# Autodesk Inventor assembly: Assembly
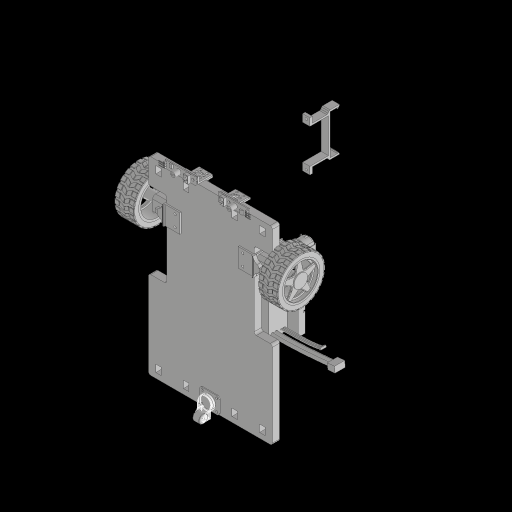
[picture p0: Inventor's stored thumbnail of the model, 512x512]
Saved by Autodesk Inventor 2024.3 (Build 283343010, 343A)
## iProperties
Created: 2025-04-09
Part Number: Assembly
Document SubType Name: Assembly
Designer: Oleg Kelner
Author: Oleg Kelner
## Documents named in this file (14)
- D:\Study\Prototyping\Prototyping-SS25-Team-C4\3DModels\Assembly.iam
- D:\Study\Prototyping\Prototyping-SS25-Team-C4\3DModels\Basic components\chassis.ipt
- D:\Study\Prototyping\Prototyping-SS25-Team-C4\3DModels\Basic components\motor-with-tire.ipt
- D:\Study\Prototyping\Prototyping-SS25-Team-C4\3DModels\Basic components\front-wheel.ipt
- D:\Study\Prototyping\Prototyping-SS25-Team-C4\3DModels\Basic components\motor-with-tire_MIR.ipt
- D:\Study\Prototyping\Prototyping-SS25-Team-C4\3DModels\Basic components\lipo-battery.ipt
- D:\Study\Prototyping\Prototyping-SS25-Team-C4\3DModels\Basic components\arduino.ipt
- D:\Study\Prototyping\Prototyping-SS25-Team-C4\3DModels\Basic components\breadboard.ipt
- D:\Study\Prototyping\Prototyping-SS25-Team-C4\3DModels\Basic components\motorcontroler.ipt
- D:\Study\Prototyping\Prototyping-SS25-Team-C4\3DModels\Oleg's details\vertMotorHolder.ipt
- D:\Study\Prototyping\Prototyping-SS25-Team-C4\3DModels\Oleg's details\batteryHolder.ipt
- D:\Work\HSHL\Kart\Kart Assembly Parts\infrared-sensor-new.ipt
- D:\Study\Prototyping\Prototyping-SS25-Team-C4\3DModels\Details to print\IRsensorHolder.ipt
- D:\Study\Prototyping\Prototyping-SS25-Team-C4\3DModels\Details to print\IRsensorHolder2.ipt
## Components (18 placed, 13 different names)
1. chassis:1 — Rigid:1, Rigid:2, Rigid:3, Slider:1, Planar:1, Angle:1, Flush:1, Mate:1, Flush:2, Mate:3, Flush:5, Flush:6
2. motor-with-tire:1 — Rotational:11, Rotational:12
3. front-wheel:1 — Rigid:1
4. motor-with-tire_MIR:1 — Rotational:9, Rotational:10
5. lipo-battery:1 — Slider:1, Rigid:4, Rigid:5
6. arduino:1
7. breadboard:1 — Rigid:5
8. motorcontroler:1
9. vertMotorHolder:1 — Rigid:3, Mate:2, Rotational:11, Rotational:12
10. vertMotorHolder:2 — Rigid:2, Rotational:9, Rotational:10
11. batteryHolder:1 — Mate:2, Rigid:4
12. batteryHolder:2
13. infrared-sensor-new:1 — Rotational:5, Rotational:6
14. IRsensorHolder:1 — Planar:1, Angle:1, Rotational:5, Rotational:6, Flush:1, Slider:2
15. IRsensorHolder2:1 — Slider:2, Mate:1, Flush:2
16. infrared-sensor-new:2 — Rotational:7, Rotational:8
17. IRsensorHolder:2 — Rotational:7, Rotational:8, Slider:3
18. IRsensorHolder2:2 — Slider:3, Mate:3, Flush:5, Flush:6
## Relationships (25: RevoluteJoint 8, WeldJoint 5, Flush 4, TranslationJoint 3, Mate 3, PlanarJoint 1, Angle 1)
- Rigid:1 [WeldJoint]: chassis:1 ↔ front-wheel:1
- Rigid:2 [WeldJoint] (-30 mm): chassis:1 ↔ vertMotorHolder:2
- Rigid:3 [WeldJoint] (30 mm): chassis:1 ↔ vertMotorHolder:1
- Slider:1 [TranslationJoint]: chassis:1 ↔ lipo-battery:1
- Planar:1: chassis:1 ↔ IRsensorHolder:1
- Angle:1 (0 deg): chassis:1 ↔ IRsensorHolder:1
- Rotational:5 [RevoluteJoint]: infrared-sensor-new:1 ↔ IRsensorHolder:1
- Rotational:6 [RevoluteJoint]: infrared-sensor-new:1 ↔ IRsensorHolder:1
- Flush:1 (-9.744 mm): chassis:1 ↔ IRsensorHolder:1
- Slider:2 [TranslationJoint]: IRsensorHolder:1 ↔ IRsensorHolder2:1
- Mate:1: chassis:1 ↔ IRsensorHolder2:1
- Flush:2 (50 mm): chassis:1 ↔ IRsensorHolder2:1
- Mate:2 (20 mm): vertMotorHolder:1 ↔ batteryHolder:1
- Rotational:7 [RevoluteJoint]: infrared-sensor-new:2 ↔ IRsensorHolder:2
- Rotational:8 [RevoluteJoint]: infrared-sensor-new:2 ↔ IRsensorHolder:2
- Slider:3 [TranslationJoint]: IRsensorHolder:2 ↔ IRsensorHolder2:2
- Mate:3: chassis:1 ↔ IRsensorHolder2:2
- Flush:5 (-50 mm): chassis:1 ↔ IRsensorHolder2:2
- Flush:6: chassis:1 ↔ IRsensorHolder2:2
- Rigid:4 [WeldJoint] (-15 mm): lipo-battery:1 ↔ batteryHolder:1
- Rigid:5 [WeldJoint] (2.5 mm): lipo-battery:1 ↔ breadboard:1
- Rotational:9 [RevoluteJoint]: motor-with-tire_MIR:1 ↔ vertMotorHolder:2
- Rotational:10 [RevoluteJoint]: motor-with-tire_MIR:1 ↔ vertMotorHolder:2
- Rotational:11 [RevoluteJoint]: motor-with-tire:1 ↔ vertMotorHolder:1
- Rotational:12 [RevoluteJoint]: motor-with-tire:1 ↔ vertMotorHolder:1
## Named parameters: d96_d82 = 0 mm, d97_d83 = 90 deg, d98_d84 = 0 mm, d99_d85 = 180 deg, d100_d91 = 0 mm, d101_d92 = 0.5 mm
